# Autodesk Inventor assembly: Motherboard_assembly
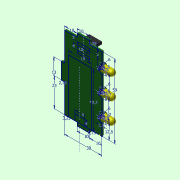
[picture p0: Inventor's stored thumbnail of the model, 180x180]
Saved by Autodesk Inventor 2015 (Build 190159000, 159)
## iProperties
Created: 2015-06-12
Part Number: Motherboard_assembly
Document SubType Name: Assembly
Designer: Openlab
Author: Openlab
## Documents named in this file (3)
- D:\Alexey\HS-Spectrophotometer\parts\Motherboard_assembly.iam
- D:\Alexey\HS-Spectrophotometer\parts\Motherboard_dummy.ipt
- D:\Alexey\HS-Spectrophotometer\parts\LED.ipt
## Components (4 placed, 2 different names)
1. Motherboard_dummy:1 — Mate:1, Mate:2, Mate:3, Mate:4, Mate:5, Mate:6, Mate:7, Mate:8, Mate:9
2. LED:1 — Mate:1, Mate:2, Mate:3
3. LED:2 — Mate:4, Mate:5, Mate:6
4. LED:3 — Mate:7, Mate:8, Mate:9
## Relationships (9: Mate 9)
- Mate:1: Motherboard_dummy:1 ↔ LED:1
- Mate:2: Motherboard_dummy:1 ↔ LED:1
- Mate:3: Motherboard_dummy:1 ↔ LED:1
- Mate:4: Motherboard_dummy:1 ↔ LED:2
- Mate:5: Motherboard_dummy:1 ↔ LED:2
- Mate:6: Motherboard_dummy:1 ↔ LED:2
- Mate:7: Motherboard_dummy:1 ↔ LED:3
- Mate:8: Motherboard_dummy:1 ↔ LED:3
- Mate:9: Motherboard_dummy:1 ↔ LED:3
